(part 1 of 2)
# Autodesk Inventor assembly: HCMUTE-CDT23-PLXR_ASEMBLY
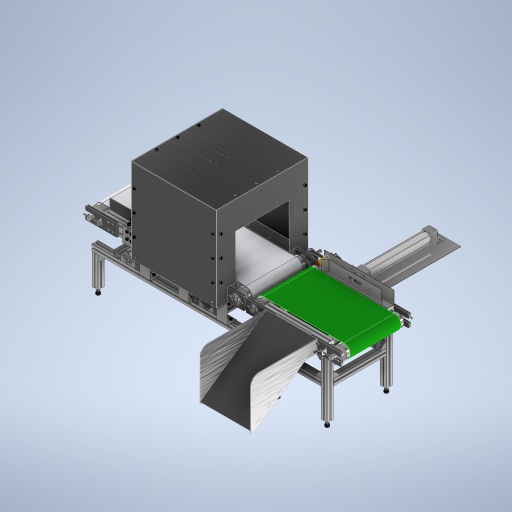
[picture p0: Inventor's stored thumbnail of the model, 512x512]
Saved by Autodesk Inventor 2023 (Build 270158000, 158)
## iProperties
Created: 2023-11-19
Part Number: HCMUTE-CDT23-PLXR_ASEMBLY
Document SubType Name: Assembly
Designer: havie
Mass: 52555 g
Surface Area: 83477.5 cm^2
Volume: 13075.1 cm^3
Density: 4.01946 g/cm^3
Author: havie
## Documents named in this file (82)
- D:\DO_AN_CDT\1.1. PART\HCMUTE-CDT23-PLXR_ASEMBLY.iam
- D:\DO_AN_CDT\1.1. PART\HCMUTE-CDT23-FRAME_ASEMBLY.iam
- D:\DO_AN_CDT\1.1. PART\HCMUTE-CDT23-BAT_TRUC_DAN.ipt
- C:\Users\havie\Documents\Inventor\Content Center Files\R2023\en-US\ISO 4762(2)\ISO 4762 - M6 x 16ISO.ipt
- D:\DO_AN_CDT\1.1. PART\HCMUTE-CDT23-GOI_DO_KFL003.ipt
- D:\DO_AN_CDT\1.1. PART\HCMUTE-CDT23-TRUC_DAN.ipt
- D:\DO_AN_CDT\1.1. PART\HCMUTE-CDT23-BAT_CANG_BANG_TAI.ipt
- D:\DO_AN_CDT\1.1. PART\HCMUTE-CDT23-BAT_TRUC_CANG_TAI.ipt
- C:\Users\havie\Documents\Inventor\Content Center Files\R2023\en-US\ISO 4762(2)\ISO 4762 - M6 x 20ISO.ipt
- D:\DO_AN_CDT\1.1. PART\HCMUTE-CDT23-TRUC_CANG.ipt
- D:\DO_AN_CDT\1.1. PART\HCMUTE-CDT23-M6X80_SUOT.ipt
- C:\Users\havie\Documents\Inventor\Content Center Files\R2023\en-US\ISO 7092\ISO 7092 - ST 6 - 140 HV.ipt
- C:\Users\havie\Documents\Inventor\Content Center Files\R2023\en-US\ISO 4032(2)\ISO 4032 - M6 - ISO.ipt
- D:\DO_AN_CDT\1.1. PART\HCMUTE-CDT23-BELT_PHAN_LOAI.ipt
- C:\Users\havie\Documents\Inventor\Content Center Files\R2023\en-US\ISO 4762(2)\ISO 4762 - M6 x 25ISO.ipt
- C:\Users\havie\Documents\Inventor\Content Center Files\R2023\en-US\ISO 4034(2)\ISO 4034 - M6 - ISO.ipt
- D:\DO_AN_CDT\1.1. PART\HCMUTE-CDT23-LOADCELL.ipt
- D:\DO_AN_CDT\1.1. PART\HCMUTE-CDT23-DE_CHEM_LOADCELL.ipt
- D:\DO_AN_CDT\1.1. PART\HCMUTE-CDT23-DE_GA_LOADCELL.ipt
- D:\DO_AN_CDT\1.1. PART\HCMUTE-CDT23-GOI_CHONG_QTAI.ipt
- D:\DO_AN_CDT\1.1. PART\HCMUTE-CDT23-GOI_DO.ipt
- C:\Users\havie\Documents\Inventor\Content Center Files\R2023\en-US\ISO 4017(1)\ISO 4017 - M6 x 45 - ISO.ipt
- C:\Users\havie\Documents\Inventor\Content Center Files\R2023\en-US\ISO 4762(2)\ISO 4762 - M6 x 10ISO.ipt
- D:\DO_AN_CDT\1.1. PART\HCMUTE-CDT23-BAN_CAN_LOADCELL.ipt
- D:\DO_AN_CDT\1.1. PART\BANG_TAI_CAN\HCMUTE-CDT23-BTC_ASEMBLY.iam
- C:\Users\havie\Documents\Inventor\Content Center Files\R2023\en-US\ISO 4762(2)\ISO 4762 - M5 x 10ISO.ipt
- C:\Users\havie\Documents\Inventor\Content Center Files\R2023\en-US\ISO 4034(2)\ISO 4034 - M5 - ISO.ipt
- D:\DO_AN_CDT\1.1. PART\HCMUTE-CDT23-PULLY_S5M-15X15X8.ipt
- D:\DO_AN_CDT\1.1. PART\HCMUTE-CDT23-PULLY_S5M-30X15X12.ipt
- D:\DO_AN_CDT\1.1. PART\2309HCMUTE-CDT23-BELT_S5M-320X64X15.ipt
- D:\DO_AN_CDT\1.1. PART\HCMUTE-CDT23-MOTOR_DC24V-100RPM-XD42GA775.ipt
- D:\DO_AN_CDT\1.1. PART\2309HCMUTE-CDT23-BELT_S5M-355X71X15.ipt
- D:\DO_AN_CDT\1.1. PART\HCMUTE-CDT23-GA_DC.ipt
- D:\DO_AN_CDT\1.1. PART\HCMUTE-CDT23-OP_GA-CONLAN.ipt
- D:\DO_AN_CDT\1.1. PART\HCMUTE-CDT23-OP_GA-STEP-42.ipt
- D:\DO_AN_CDT\1.1. PART\HCMUTE-CDT23-OP_NDH-2020X500.ipt
- D:\DO_AN_CDT\1.1. PART\HCMUTE-CDT23-OP_STEP-42.ipt
- C:\Users\havie\Documents\Inventor\Content Center Files\R2023\en-US\ISO 4762(2)\ISO 4762 - M6 x 12ISO.ipt
- C:\Users\havie\Documents\Inventor\Content Center Files\R2023\en-US\301818\301818.ipt
- D:\DO_AN_CDT\1.1. PART\HCMUTE-CDT23-OP_TAMLOT.ipt
- C:\Users\havie\Documents\Inventor\Content Center Files\R2023\en-US\ISO 4762(2)\ISO 4762 - M5 x 12ISO.ipt
- D:\DO_AN_CDT\1.1. PART\HCMUTE-CDT23-OP_PULLY-GT2-30X6X5.ipt
- C:\Users\havie\Documents\Inventor\Content Center Files\R2023\en-US\ISO 4762(2)\ISO 4762 - M5 x 8ISO.ipt
- D:\DO_AN_CDT\1.1. PART\HCMUTE-CDT23-OP_RONG-ROC.ipt
- D:\DO_AN_CDT\1.1. PART\HCMUTE-CDT23-OP_V-WHEEL.ipt
- D:\DO_AN_CDT\1.1. PART\HCMUTE-CDT23-OP_BASE-PLATE.ipt
- D:\DO_AN_CDT\1.1. PART\HCMUTE-CDT23-OP_DVCAM.ipt
- D:\DO_AN_CDT\1.1. PART\CAMERA\Assembly_HCMUTE-CDT23-CAMERA_C270Logitech c270 Assembly.iam
- D:\DO_AN_CDT\1.1. PART\HCMUTE-CDT23-OP_RONG-ROC2.ipt
- D:\DO_AN_CDT\1.1. PART\HCMUTE-CDT23-KXL_CHAN-GA.ipt
- D:\DO_AN_CDT\1.1. PART\HCMUTE-CDT23-KXL_A01.ipt
- C:\Users\havie\Documents\Inventor\Content Center Files\R2023\en-US\ISO 4032(2)\ISO 4032 - M5 - ISO.ipt
- D:\DO_AN_CDT\1.1. PART\2309HCMUTE-CDT23-KXL_GA-VUONG.ipt
- D:\DO_AN_CDT\1.1. PART\HCMUTE-CDT23-KXL_A02.ipt
- D:\DO_AN_CDT\1.1. PART\HCMUTE-CDT23-KXL_A03.ipt
- D:\DO_AN_CDT\1.1. PART\HCMUTE-CDT23-KXL_A04.ipt
- D:\DO_AN_CDT\1.1. PART\HCMUTE-CDT23-KXL_A05.ipt
- D:\DO_AN_CDT\1.1. PART\Part_Cylinder\Assembly_HCMUTE-CDT23-CYLINDER-AIRTAC_SC32X300.iam
- D:\DO_AN_CDT\1.1. PART\HCMUTE-CDT23-TAY_GAT.ipt
- D:\DO_AN_CDT\1.1. PART\Part_Cylinder\2309HCMUTE-CDT23-BE_DO.ipt
- D:\DO_AN_CDT\1.1. PART\HCMUTE-CDT23-VND.ipt
- D:\DO_AN_CDT\1.1. PART\Part_Cylinder\2309HCMUTE-CDT23-DO_GA.ipt
- D:\DO_AN_CDT\1.1. PART\HCMUTE-CDT23-BAC_TRUOT.ipt
- D:\DO_AN_CDT\1.1. PART\HCMUTE-CDT23-TRUC_TRUOT.ipt
- D:\DO_AN_CDT\1.1. PART\CBIEN\Assembly_HCMUTE-CDT23-CB_E3F-DS30C4.iam
- D:\DO_AN_CDT\1.1. PART\Part_Contain-Sample\Assembly_HCMUTE-CDT23_BE-TRUOT.iam
- D:\DO_AN_CDT\1.1. PART\HCMUTE-CDT23-BTC-VND.ipt
- D:\DO_AN_CDT\1.1. PART\HCMUTE-CDT23-OP_GA-CONLAN3.ipt
- D:\DO_AN_CDT\1.1. PART\HCMUTE-CDT23-OP_GA-STEP-423.ipt
- D:\DO_AN_CDT\1.1. PART\HCMUTE-CDT23-OP_NDH-2020X5003.ipt
- D:\DO_AN_CDT\1.1. PART\HCMUTE-CDT23-OP_STEP-423.ipt
- D:\DO_AN_CDT\1.1. PART\HCMUTE-CDT23-OP_TAMLOT3.ipt
- D:\DO_AN_CDT\1.1. PART\HCMUTE-CDT23-OP_PULLY-GT2-30X6X53.ipt
- D:\DO_AN_CDT\1.1. PART\HCMUTE-CDT23-OP_RONG-ROC3.ipt
- D:\DO_AN_CDT\1.1. PART\HCMUTE-CDT23-OP_V-WHEEL1.ipt
- D:\DO_AN_CDT\1.1. PART\HCMUTE-CDT23-OP_BASE-PLATE3.ipt
- D:\DO_AN_CDT\1.1. PART\2309HCMUTE-CDT23-KXL_GA-VUONG1.ipt
- D:\DO_AN_CDT\1.1. PART\HCMUTE-CDT23-KXL_A06.ipt
- C:\Users\havie\Documents\Inventor\Content Center Files\R2023\en-US\ISO 4762(2)\ISO 4762 - M4 x 16ISO.ipt
- C:\Users\havie\Documents\Inventor\Content Center Files\R2023\en-US\ISO 4032(2)\ISO 4032 - M4 - ISO.ipt
- D:\DO_AN_CDT\1.1. PART\BANG_TAI_CAN\HCMUTE-CDT23-GOI_DO_KFL003.ipt
- C:\Users\havie\Documents\Inventor\Content Center Files\R2023\en-US\302828\302828.ipt
## Components (366 placed, 80 different names)
1. HCMUTE-CDT23-FRAME_ASEMBLY:1 [sub-assembly] — Mate:1, Flush:1, Flush:2, Mate:18, Mate:19, Mate:20, Mate:21, Flush:5, Mate:33, Mate:35, Mate:36, Mate:37, Mate:38, Mate:40, Mate:42, Flush:6, Mate:73, Mate:84, Flush:8, Flush:9, Mate:92, Flush:12, Mate:102, Flush:13, Mate:152, Flush:16, Mate:153, Flush:18, Mate:154, Flush:20, Mate:185, Mate:186, Mate:190, Mate:206, Flush:30, Flush:32, Flush:35, Mate:276, Flush:52, Mate:277, Mate:282, Mate:283, Mate:284, Mate:285, Mate:320, Flush:63, Mate:321, Mate:322, Mate:323, Mate:399, Flush:73, Mate:402, Mate:498, Mate:499, Flush:96, Mate:500, Mate:501, Flush:97, Mate:502, Mate:503, Flush:98, Mate:504, Mate:505, Flush:99
2. HCMUTE-CDT23-BAT_TRUC_DAN:1 — Mate:1, Flush:1, Flush:2, Mate:7, Mate:8, Mate:9, Mate:74, Mate:75, Mate:76, Mate:77, Mate:194, Mate:196
3. HCMUTE-CDT23-BAT_TRUC_DAN:2 — Mate:190, Mate:191, Mate:192, Mate:193
4. HCMUTE-CDT23-GOI_DO_KFL003:1 — Mate:7, Mate:8, Mate:9, Mate:16, Mate:17, Mate:78, Mate:80
5. HCMUTE-CDT23-GOI_DO_KFL003:2 — Mate:173, Mate:191
6. HCMUTE-CDT23-BAT_CANG_BANG_TAI:1 — Mate:18, Mate:19, Mate:20, Mate:22, Mate:31, Mate:32, Mate:34, Mate:67, Mate:68, Mate:70
7. HCMUTE-CDT23-TRUC_DAN:1 — Mate:16, Mate:17, Mate:72, Mate:155, Mate:172, Mate:174, Mate:189
8. HCMUTE-CDT23-BAT_TRUC_CANG_TAI:1 — Mate:21, Flush:5, Mate:22, Mate:27, Mate:28, Mate:29, Mate:30, Mate:415, Mate:416, Mate:419, Mate:422
9. ISO 4762 M6 x 16:14 — Mate:29, Mate:30
10. ISO 4762 M6 x 16:16 — Mate:27, Mate:28
11. ISO 4762 M6 x 20:1 — Mate:31, Mate:32
12. ISO 4762 M6 x 20:2 — Mate:33, Mate:34
13. HCMUTE-CDT23-BAT_CANG_BANG_TAI:2 — Mate:35, Mate:36, Mate:37, Mate:39, Mate:41, Mate:43, Angle:1, Mate:54, Mate:56, Mate:61, Flush:77
14. ISO 4762 M6 x 20:3 — Mate:38, Mate:39
15. ISO 4762 M6 x 20:4 — Mate:40, Mate:41
16. HCMUTE-CDT23-BAT_TRUC_CANG_TAI:2 — Mate:42, Flush:6, Mate:43, Mate:44, Mate:45, Mate:46, Mate:47, Mate:48, Mate:49, Mate:50, Mate:51, Mate:52, Mate:400
17. ISO 4762 M6 x 16:17 — Mate:44, Mate:50
18. ISO 4762 M6 x 16:18 — Mate:45, Mate:51
19. ISO 4762 M6 x 16:19 — Mate:46, Mate:49
20. ISO 4762 M6 x 16:20 — Mate:47, Mate:48
21. HCMUTE-CDT23-TRUC_CANG:1 — Mate:52, Flush:7, Mate:422
22. HCMUTE-CDT23-M6X80_SUOT:1 — Mate:54, Mate:55, Mate:57, Mate:59, Mate:60
23. ISO 7092 ST 6 - 140 HV:1 — Mate:55, Mate:56, Mate:58
24. ISO 4032 M6:1 — Mate:57, Mate:58, Mate:59
25. ISO 4032 M6:2 — Mate:60, Mate:61
26. HCMUTE-CDT23-M6X80_SUOT:2 — Mate:67, Mate:69
27. ISO 7092 ST 6 - 140 HV:2 — Mate:68
28. ISO 4032 M6:3
29. ISO 4032 M6:5 — Mate:69, Mate:70
30. HCMUTE-CDT23-BELT_PHAN_LOAI:1 — Mate:72, Mate:73
31. ISO 4762 M6 x 25:1 — Mate:74, Mate:75, Mate:79
32. ISO 4762 M6 x 25:2 — Mate:76, Mate:77, Mate:81
33. ISO 4034 M6:1 — Mate:80, Mate:81
34. ISO 4034 M6:2 — Mate:78, Mate:79
35. ISO 4762 M6 x 25:3 — Mate:83, Mate:192
36. ISO 4762 M6 x 25:4 — Mate:82, Mate:193
37. ISO 4034 M6:3 — Mate:82
38. ISO 4034 M6:4 — Mate:83
39. HCMUTE-CDT23-LOADCELL:1 — Mate:88, Mate:89, Mate:90, Mate:94, Mate:95, Mate:96, Mate:97, Flush:14, Mate:113, Mate:114, Mate:115
40. HCMUTE-CDT23-DE_CHEM_LOADCELL:1 — Mate:85, Mate:86, Mate:87, Mate:88, Mate:89, Mate:90
41. HCMUTE-CDT23-DE_GA_LOADCELL:1 — Mate:84, Flush:8, Flush:9, Mate:85, Mate:86, Mate:87, Mate:93, Mate:98, Mate:99, Mate:100, Mate:101, Flush:19
42. HCMUTE-CDT23-GOI_CHONG_QTAI:1 — Mate:102, Flush:13, Mate:103, Mate:104, Flush:14
43. HCMUTE-CDT23-GOI_DO:1 — Mate:92, Flush:12, Mate:93, Mate:105, Mate:106, Mate:107, Mate:108, Mate:109, Mate:110, Mate:111, Mate:112, Flush:17
44. ISO 4017 M6 x 45:1 — Mate:94, Mate:97
45. ISO 4017 M6 x 45:2 — Mate:95, Mate:96
46. ISO 4762 M6 x 16:31 — Mate:100, Mate:101
47. ISO 4762 M6 x 16:33 — Mate:98, Mate:99
48. ISO 4762 M6 x 16:34 — Mate:103, Mate:104
49. ISO 4762 M6 x 10:1 — Mate:105, Mate:106
50. ISO 4762 M6 x 10:2 — Mate:111, Mate:112
51. ISO 4762 M6 x 10:3 — Mate:109, Mate:110
52. ISO 4762 M6 x 10:4 — Mate:107, Mate:108
53. HCMUTE-CDT23-BAN_CAN_LOADCELL:1 — Mate:113, Mate:114, Mate:115, Mate:116, Mate:117, Mate:118, Mate:119, Mate:156, Mate:157, Mate:158, Mate:159, Mate:160, Mate:161, Mate:162, Mate:163
54. ISO 4762 M6 x 25:5 — Mate:116, Mate:118
55. ISO 4762 M6 x 25:6 — Mate:117, Mate:119
56. HCMUTE-CDT23-LOADCELL:2 — Flush:21
57. HCMUTE-CDT23-DE_CHEM_LOADCELL:2
58. HCMUTE-CDT23-DE_GA_LOADCELL:2 — Mate:153, Flush:18, Flush:19
59. HCMUTE-CDT23-GOI_CHONG_QTAI:2 — Mate:154, Flush:20, Flush:21
60. HCMUTE-CDT23-GOI_DO:2 — Mate:152, Flush:16, Flush:17
61. ISO 4017 M6 x 45:3
62. ISO 4017 M6 x 45:4
63. ISO 4762 M6 x 16:35
64. ISO 4762 M6 x 16:36
65. ISO 4762 M6 x 16:37
66. ISO 4762 M6 x 10:5
67. ISO 4762 M6 x 10:6
68. ISO 4762 M6 x 10:7
69. ISO 4762 M6 x 10:8
70. HCMUTE-CDT23-BAN_CAN_LOADCELL:2
71. ISO 4762 M6 x 25:7
72. ISO 4762 M6 x 25:8
73. HCMUTE-CDT23-BTC_ASEMBLY:1 [sub-assembly] — Mate:155, Mate:164, Mate:166, Mate:168, Mate:170, Mate:176, Mate:178, Mate:203, Mate:423, Flush:78, Mate:425, Mate:426, Flush:92, Mate:462, Flush:93, Flush:95, Mate:497
74. HCMUTE-CDT23-PULLY_S5M-30X15X12:1 — Mate:172, Mate:173, Mate:175, Flush:24, Mate:177, Mate:179
75. HCMUTE-CDT23-PULLY_S5M-30X15X12:2 — Mate:174, Mate:175, Flush:25
76. HCMUTE-CDT23-PULLY_S5M-30X15X12:3 — Mate:176, Flush:24
77. 2309HCMUTE-CDT23-BELT_S5M-320X64X15:1 — Mate:177, Mate:178, Mate:179
78. HCMUTE-CDT23-MOTOR_DC24V-100RPM-XD42GA775:1 — Mate:180, Mate:181, Mate:182, Mate:183
79. HCMUTE-CDT23-PULLY_S5M-15X15X8:1 — Mate:183, Mate:184, Flush:25, Mate:187, Mate:188
80. 2309HCMUTE-CDT23-BELT_S5M-355X71X15:1 — Mate:187, Mate:188, Mate:189
81. HCMUTE-CDT23-GA_DC:1 — Mate:180, Mate:181, Mate:182, Mate:184, Mate:185, Mate:186
82. HCMUTE-CDT23-OP_GA-CONLAN:1 — Mate:202, Flush:28, Flush:34, Mate:221, Mate:222, Mate:223, Mate:224, Mate:225, Mate:226, Mate:236
83. HCMUTE-CDT23-OP_GA-STEP-42:1 — Mate:199, Flush:26, Flush:27, Mate:200, Mate:201, Mate:216, Mate:217, Mate:218, Mate:219, Mate:220
84. HCMUTE-CDT23-OP_NDH-2020X500:1 — Mate:199, Flush:26, Flush:27, Mate:202, Flush:28, Mate:203, Flush:31, Mate:208, Mate:210, Flush:34, Flush:35, Flush:39, Flush:40, Mate:426, Flush:80
85. HCMUTE-CDT23-OP_STEP-42:1 — Mate:200, Mate:201, Mate:215
86. ISO 4762 M6 x 12:7
87. ISO 4762 M6 x 12:8
88. ISO 4762 M6 x 12:9
89. ISO 4762 M6 x 12:10
90. ISO 4762 M6 x 12:11
91. ISO 4762 M6 x 12:12
92. 301818 302828.1:1 — Mate:207, Mate:208, Flush:32, Flush:33, Mate:214
93. HCMUTE-CDT23-OP_TAMLOT:1 — Mate:206, Flush:30, Flush:31, Mate:207, Mate:209, Mate:211, Mate:213
94. 301818 302828.1:2 — Mate:209, Mate:210, Flush:33, Mate:212
95. ISO 4762 M5 x 12:1 — Mate:211, Mate:212
96. ISO 4762 M5 x 12:2 — Mate:213, Mate:214
97. HCMUTE-CDT23-OP_PULLY-GT2-30X6X5:1 — Mate:215, Mate:216
98. ISO 4762 M5 x 8:1 — Mate:217, Mate:218
99. ISO 4762 M5 x 8:2 — Mate:219, Mate:220
100. ISO 4762 M5 x 8:3 — Mate:221, Mate:222
101. ISO 4762 M5 x 8:4 — Mate:223, Mate:224
102. HCMUTE-CDT23-OP_RONG-ROC:1 — Mate:225, Mate:226
103. HCMUTE-CDT23-OP_V-WHEEL:1 — Mate:227, Mate:228, Flush:37, Flush:38
104. HCMUTE-CDT23-OP_BASE-PLATE:1 — Mate:227, Mate:228, Mate:229, Mate:230, Mate:231, Mate:232, Mate:233, Mate:234, Angle:3, Mate:236, Flush:80, Mate:427, Mate:428, Angle:9
105. HCMUTE-CDT23-OP_V-WHEEL:3 — Mate:229, Mate:230
106. HCMUTE-CDT23-OP_V-WHEEL:4 — Mate:231, Mate:232
107. HCMUTE-CDT23-OP_V-WHEEL:5 — Mate:233, Mate:234
108. HCMUTE-CDT23-OP_DVCAM:1 — Mate:273, Mate:274, Mate:275, Mate:427, Mate:428, Angle:9
109. Assembly_HCMUTE-CDT23-CAMERA_C270Logitech c270 Assembly:1 [sub-assembly] — Mate:273, Mate:274, Mate:275
110. HCMUTE-CDT23-OP_RONG-ROC2:1
111. HCMUTE-CDT23-KXL_CHAN-GA:1 — Mate:276, Flush:52, Mate:277, Mate:278, Mate:279, Mate:280, Mate:281, Flush:53, Mate:286, Mate:287
112. HCMUTE-CDT23-KXL_CHAN-GA:2 — Mate:282, Mate:283, Flush:53, Flush:54, Flush:65
113. HCMUTE-CDT23-KXL_CHAN-GA:3 — Mate:284, Mate:285, Flush:54, Mate:296, Flush:67
114. HCMUTE-CDT23-KXL_A01:1 — Mate:286, Mate:287, Mate:288, Flush:55, Mate:289, Mate:290, Mate:291, Mate:292, Mate:293, Flush:57, Mate:313, Mate:360
115. 2309HCMUTE-CDT23-KXL_GA-VUONG:1 — Mate:288, Flush:55, Mate:289, Flush:56, Mate:476, Mate:477
116. 2309HCMUTE-CDT23-KXL_GA-VUONG:2 — Mate:290, Flush:56, Mate:291
117. 2309HCMUTE-CDT23-KXL_GA-VUONG:3 — Mate:292, Mate:293, Flush:57, Mate:478
118. ISO 4032 M5:1 — Mate:296
119. HCMUTE-CDT23-KXL_A03:1 — Mate:313, Mate:316, Mate:319, Flush:61, Flush:62, Mate:338, Mate:355, Mate:356, Mate:370, Symmetry:3
120. HCMUTE-CDT23-KXL_A02:2 — Mate:319, Flush:61, Flush:62, Mate:333, Mate:334, Mate:335, Flush:69, Mate:336, Mate:337, Mate:341, Mate:342, Mate:347, Mate:348, Mate:351, Mate:352, Mate:474, Mate:475
121. HCMUTE-CDT23-KXL_CHAN-GA:4 — Mate:320, Flush:63, Mate:321, Flush:64, Flush:66
122. HCMUTE-CDT23-KXL_CHAN-GA:5 — Mate:322, Flush:64, Flush:65, Mate:326
123. HCMUTE-CDT23-KXL_CHAN-GA:6 — Mate:323, Flush:66, Flush:67, Mate:324, Flush:68, Mate:325, Mate:327, Mate:328, Mate:329, Mate:330, Mate:332, Mate:340
124. HCMUTE-CDT23-KXL_A01:2 — Mate:324, Flush:68, Mate:325, Mate:326, Mate:331
125. HCMUTE-CDT23-KXL_A04:1 — Mate:360, Mate:361, Mate:362, Mate:363, Mate:364, Mate:373, Mate:380, Mate:381, Symmetry:3
126. HCMUTE-CDT23-KXL_A05:1 — Mate:370, Mate:371, Flush:72, Mate:372, Mate:374, Mate:375, Mate:382, Mate:383, Mate:384, Mate:385, Mate:386, Mate:481, Mate:482, Mate:483, Mate:484, Mate:485, Mate:486, Mate:487, Mate:488
127. ISO 4762 M5 x 12:44
128. ISO 4032 M5:40
129. ISO 4032 M5:41
130. ISO 4762 M5 x 12:45
131. ISO 4762 M5 x 12:46
132. ISO 4032 M5:42
133. ISO 4032 M5:43
134. ISO 4762 M5 x 12:47
135. ISO 4762 M5 x 12:48
136. ISO 4032 M5:44
137. ISO 4032 M5:45
138. ISO 4762 M5 x 12:49
139. Assembly_HCMUTE-CDT23-CAMERA_C270Logitech c270 Assembly:2 [sub-assembly] — Mate:384, Mate:385, Mate:386, Mate:493, Mate:494, Mate:495, Mate:496
140. Assembly_HCMUTE-CDT23-CYLINDER-AIRTAC_SC32X300:1 [sub-assembly] — Tangent:1, Mate:401, Mate:403, Mate:404, Angle:6, Mate:405, Mate:406, Mate:407
141. HCMUTE-CDT23-TAY_GAT:1 — Tangent:1, Mate:401, Flush:76, Mate:412
142. 2309HCMUTE-CDT23-BE_DO:1 — Mate:399, Flush:73, Mate:400, Flush:74
143. HCMUTE-CDT23-VND:1 — Mate:402, Flush:74, Mate:403, Mate:404, Angle:6, Mate:408, Mate:409, Mate:410, Flush:77, Mate:413, Mate:414
144. 2309HCMUTE-CDT23-DO_GA:1 — Mate:405, Mate:406, Mate:407
145. HCMUTE-CDT23-BAC_TRUOT:1 — Mate:408, Mate:409, Mate:410, Mate:411
146. HCMUTE-CDT23-TRUC_TRUOT:1 — Mate:411, Flush:76, Mate:412
147. Assembly_HCMUTE-CDT23-CB_E3F-DS30C4:1 [sub-assembly] — Mate:413, Mate:414
148. Assembly_HCMUTE-CDT23_BE-TRUOT:1 [sub-assembly] — Angle:7, Angle:8, Mate:415, Mate:416, Mate:417, Mate:418, Mate:419, Mate:420, Mate:421
149. ISO 4762 M6 x 16:38 — Mate:417, Mate:418
150. ISO 4762 M6 x 16:39 — Mate:420, Mate:421
151. HCMUTE-CDT23-BTC-VND:1 — Mate:424, Mate:425, Flush:92, Flush:94, Mate:468
152. HCMUTE-CDT23-OP_GA-CONLAN3:1 — Flush:81, Flush:82, Mate:429, Mate:447, Mate:449, Mate:451, Mate:452, Mate:453
153. HCMUTE-CDT23-OP_GA-STEP-423:1 — Flush:83, Flush:84, Mate:430, Mate:431, Mate:432, Mate:441, Mate:443, Mate:445
154. HCMUTE-CDT23-OP_NDH-2020X5003:1 — Flush:81, Flush:82, Mate:429, Flush:83, Flush:84, Mate:430, Mate:433, Flush:85, Mate:435, Flush:87, Flush:90, Flush:91
155. HCMUTE-CDT23-OP_STEP-423:1 — Mate:431, Mate:432, Mate:442
156. 301818 302828.1:3 — Mate:433, Mate:434, Flush:86, Mate:439
157. HCMUTE-CDT23-OP_TAMLOT3:1 — Mate:434, Flush:85, Mate:436
158. 301818 302828.1:4 — Flush:86, Mate:435, Mate:436, Mate:437
159. ISO 4762 M5 x 12:50 — Mate:437
160. ISO 4762 M5 x 12:51 — Mate:439
161. HCMUTE-CDT23-OP_PULLY-GT2-30X6X53:1 — Mate:441, Mate:442
162. ISO 4762 M5 x 8:5 — Mate:443
163. ISO 4762 M5 x 8:6 — Mate:445
164. ISO 4762 M5 x 8:7 — Mate:447
165. ISO 4762 M5 x 8:8 — Mate:449
166. HCMUTE-CDT23-OP_RONG-ROC3:1 — Mate:451, Mate:452
167. HCMUTE-CDT23-OP_V-WHEEL1:1 — Mate:454, Mate:455, Flush:88, Flush:89
168. HCMUTE-CDT23-OP_BASE-PLATE3:1 — Flush:87, Mate:453, Angle:10, Mate:454, Mate:455, Mate:456, Mate:457, Mate:458, Mate:459, Mate:460, Mate:461
169. HCMUTE-CDT23-OP_V-WHEEL1:2 — Mate:456, Mate:457
170. HCMUTE-CDT23-OP_V-WHEEL1:3 — Mate:458, Mate:459
171. HCMUTE-CDT23-OP_V-WHEEL1:4 — Mate:460, Mate:461
172. HCMUTE-CDT23-BTC-VND:2 — Mate:462, Flush:93, Flush:94
173. 2309HCMUTE-CDT23-KXL_GA-VUONG1:1 — Mate:469, Mate:471
174. 2309HCMUTE-CDT23-KXL_GA-VUONG1:2
175. 2309HCMUTE-CDT23-KXL_GA-VUONG1:3
176. 2309HCMUTE-CDT23-KXL_GA-VUONG1:4
177. 2309HCMUTE-CDT23-KXL_GA-VUONG1:5
178. ISO 4762 M5 x 12:62 — Mate:471, Mate:473
179. ISO 4032 M5:51 — Mate:473
180. ISO 4762 M5 x 12:63 — Mate:469
181. ISO 4762 M5 x 12:64
182. ISO 4032 M5:52
183. ISO 4762 M5 x 12:65
184. ISO 4762 M5 x 12:66
185. ISO 4032 M5:53
186. ISO 4762 M5 x 12:67
187. ISO 4762 M5 x 12:68
188. ISO 4032 M5:54
189. ISO 4762 M5 x 12:69
190. ISO 4762 M5 x 12:70
191. ISO 4032 M5:55
192. ISO 4762 M5 x 12:71
193. Assembly_HCMUTE-CDT23-CB_E3F-DS30C4:2 [sub-assembly] — Mate:474, Mate:475
194. HCMUTE-CDT23-KXL_A06:1 — Mate:476, Mate:477, Mate:478
195. ISO 4032 M5:60 — Mate:479
196. ISO 4032 M5:61 — Mate:480
197. ISO 4762 M5 x 12:76 — Mate:480
198. ISO 4762 M5 x 12:77 — Mate:479
199. ISO 4032 M5:62
200. ISO 4032 M5:63
201. ISO 4762 M5 x 12:78
202. ISO 4762 M5 x 12:79
203. ISO 4032 M5:64
204. ISO 4032 M5:65
205. ISO 4762 M5 x 12:80
206. ISO 4762 M5 x 12:81
207. ISO 4762 M4 x 16:1 — Mate:483, Mate:486, Mate:490
208. ISO 4762 M4 x 16:2 — Mate:482, Mate:487, Mate:489
209. ISO 4762 M4 x 16:3 — Mate:481, Mate:488, Mate:491
210. ISO 4762 M4 x 16:4 — Mate:484, Mate:485, Mate:492
211. ISO 4032 M4:1 — Mate:489, Mate:494
212. ISO 4032 M4:2 — Mate:490, Mate:496
213. ISO 4032 M4:3 — Mate:491, Mate:493
214. ISO 4032 M4:4 — Mate:492, Mate:495
215. HCMUTE-CDT23-GOI_DO_KFL003:3 — Mate:497
216. 302828 302828:1 — Mate:498, Mate:499, Flush:96
217. 302828 302828:2 — Mate:500, Mate:501, Flush:97
218. 302828 302828:3 — Mate:502, Mate:503, Flush:98
219. 302828 302828:4 — Mate:504, Mate:505, Flush:99
220. ISO 4034 M5:2 — Mate:166, Mate:167
221. ISO 4762 M5 x 10:1 — Mate:156, Mate:157, Mate:167
222. ISO 4034 M5:3 — Mate:168, Mate:169
223. ISO 4762 M5 x 10:3 — Mate:160, Mate:161, Mate:169
224. ISO 4034 M5:4 — Mate:170, Mate:171
225. ISO 4034 M5:1 — Mate:164, Mate:165
226. ISO 4762 M5 x 10:4 — Mate:162, Mate:163, Mate:165
227. ISO 4762 M5 x 10:2 — Mate:158, Mate:159, Mate:171
228. ISO 4034 M5:5
229. ISO 4762 M5 x 10:5
230. ISO 4034 M5:6
231. ISO 4762 M5 x 10:6
232. ISO 4034 M5:7
233. ISO 4034 M5:8
234. ISO 4762 M5 x 10:7
235. ISO 4762 M5 x 10:8
236. ISO 4762 M6 x 12:1 — Mate:194
237. ISO 4762 M6 x 12:2 — Mate:196
238. ISO 4762 M6 x 12:3
239. ISO 4762 M6 x 12:4
240. ISO 4762 M6 x 12:5
241. ISO 4762 M6 x 12:6
242. ISO 4762 M6 x 10:9 — Mate:280, Mate:281
243. ISO 4762 M6 x 10:10 — Mate:278, Mate:279
244. ISO 4762 M6 x 10:11
245. ISO 4762 M6 x 10:12
246. ISO 4762 M6 x 10:13
247. ISO 4762 M6 x 10:14
248. ISO 4032 M5:10 — Mate:317, Mate:318
249. ISO 4762 M5 x 12:14 — Mate:315, Mate:316, Mate:318
250. ISO 4032 M5:11
251. ISO 4762 M5 x 12:15
252. ISO 4032 M5:12
253. ISO 4762 M5 x 12:16
254. ISO 4762 M6 x 10:16 — Mate:329, Mate:330
255. ISO 4762 M6 x 10:15 — Mate:327, Mate:328
256. ISO 4762 M6 x 10:17
257. ISO 4762 M6 x 10:18
258. ISO 4762 M6 x 10:19
259. ISO 4762 M6 x 10:20
260. 2309HCMUTE-CDT23-KXL_GA-VUONG:10 — Mate:331, Mate:332, Mate:333, Mate:339, Mate:343, Mate:345
261. 2309HCMUTE-CDT23-KXL_GA-VUONG:13
262. 2309HCMUTE-CDT23-KXL_GA-VUONG:14
263. 2309HCMUTE-CDT23-KXL_GA-VUONG:11 — Mate:334, Mate:335, Flush:69, Mate:349
264. 2309HCMUTE-CDT23-KXL_GA-VUONG:12 — Mate:336, Mate:337, Mate:338, Mate:354, Mate:357
265. 2309HCMUTE-CDT23-KXL_GA-VUONG:15
266. 2309HCMUTE-CDT23-KXL_GA-VUONG:16
267. 2309HCMUTE-CDT23-KXL_GA-VUONG:17 — Mate:367
268. 2309HCMUTE-CDT23-KXL_GA-VUONG:18
269. ISO 4032 M5:15 — Mate:343, Mate:344
270. ISO 4032 M5:16 — Mate:345, Mate:346
271. ISO 4762 M5 x 12:20 — Mate:341, Mate:342, Mate:346
272. ISO 4762 M5 x 12:17 — Mate:339, Mate:340, Mate:344
273. ISO 4032 M5:17
274. ISO 4032 M5:18
275. ISO 4762 M5 x 12:21
276. ISO 4762 M5 x 12:22
277. ISO 4032 M5:19
278. ISO 4032 M5:20
279. ISO 4762 M5 x 12:23
280. ISO 4762 M5 x 12:24
281. ISO 4762 M5 x 12:18 — Mate:347, Mate:348, Mate:350
282. ISO 4032 M5:14 — Mate:349, Mate:350
283. ISO 4762 M5 x 12:25
284. ISO 4032 M5:21
285. ISO 4762 M5 x 12:26
286. ISO 4032 M5:22
287. ISO 4032 M5:13 — Mate:353, Mate:354
288. ISO 4762 M5 x 12:19 — Mate:351, Mate:352, Mate:353
289. ISO 4762 M5 x 12:27 — Mate:355, Mate:356, Mate:358
290. ISO 4032 M5:23 — Mate:357, Mate:358
291. ISO 4032 M5:24
292. ISO 4762 M5 x 12:28
293. ISO 4762 M5 x 12:29
294. ISO 4032 M5:25
295. ISO 4032 M5:26
296. ISO 4762 M5 x 12:30
297. ISO 4762 M5 x 12:31
298. ISO 4032 M5:27
299. ISO 4032 M5:29 — Mate:367, Mate:368
300. ISO 4762 M5 x 12:32 — Mate:361, Mate:362, Mate:368
301. ISO 4032 M5:28 — Mate:365, Mate:366
302. ISO 4762 M5 x 12:33 — Mate:363, Mate:364, Mate:366
303. ISO 4032 M5:30
304. ISO 4762 M5 x 12:34
305. ISO 4032 M5:31
306. ISO 4762 M5 x 12:35
307. ISO 4032 M5:32
308. ISO 4762 M5 x 12:36
309. ISO 4032 M5:33
310. ISO 4762 M5 x 12:37
311. 2309HCMUTE-CDT23-KXL_GA-VUONG:19 — Mate:371, Flush:72, Mate:372
312. 2309HCMUTE-CDT23-KXL_GA-VUONG:20
313. 2309HCMUTE-CDT23-KXL_GA-VUONG:21
314. 2309HCMUTE-CDT23-KXL_GA-VUONG:22 — Mate:373, Mate:374, Mate:375, Mate:376, Mate:377, Mate:378, Mate:379
315. 2309HCMUTE-CDT23-KXL_GA-VUONG:23
316. 2309HCMUTE-CDT23-KXL_GA-VUONG:24
317. ISO 4762 M5 x 12:38 — Mate:380, Mate:381
318. ISO 4032 M5:34 — Mate:376, Mate:377
319. ISO 4032 M5:35 — Mate:378, Mate:379
320. ISO 4762 M5 x 12:39 — Mate:382, Mate:383
321. ISO 4762 M5 x 12:40
322. ISO 4032 M5:36
323. ISO 4032 M5:37
324. ISO 4762 M5 x 12:41
325. ISO 4762 M5 x 12:42
326. ISO 4032 M5:38
327. ISO 4032 M5:39
328. ISO 4762 M5 x 12:43
329. 2309HCMUTE-CDT23-KXL_GA-VUONG:25 — Mate:423, Flush:78, Mate:424, Flush:95, Mate:463, Mate:464, Mate:465, Mate:466
330. 2309HCMUTE-CDT23-KXL_GA-VUONG:26
331. 2309HCMUTE-CDT23-KXL_GA-VUONG:27
332. 2309HCMUTE-CDT23-KXL_GA-VUONG:28
333. 2309HCMUTE-CDT23-KXL_GA-VUONG:29
334. ISO 4762 M5 x 12:53 — Mate:463, Mate:464, Mate:467
335. ISO 4032 M5:46 — Mate:467, Mate:468
336. ISO 4762 M5 x 12:52 — Mate:465, Mate:466
337. ISO 4762 M5 x 12:54
338. ISO 4032 M5:47
339. ISO 4762 M5 x 12:55
340. ISO 4762 M5 x 12:56
341. ISO 4032 M5:48
342. ISO 4762 M5 x 12:57
343. ISO 4762 M5 x 12:58
344. ISO 4032 M5:49
345. ISO 4762 M5 x 12:59
346. ISO 4762 M5 x 12:60
347. ISO 4032 M5:50
348. ISO 4762 M5 x 12:61
349. 2309HCMUTE-CDT23-KXL_GA-VUONG:4 — Mate:309, Mate:365
350. ISO 4032 M5:5 — Mate:309, Mate:310
351. ISO 4762 M5 x 12:8 — Mate:310
352. 2309HCMUTE-CDT23-KXL_GA-VUONG:30
353. ISO 4032 M5:56
354. ISO 4762 M5 x 12:72
355. 2309HCMUTE-CDT23-KXL_GA-VUONG:31
356. ISO 4032 M5:57
357. ISO 4762 M5 x 12:73
358. ISO 4032 M5:4 — Mate:311, Mate:312
359. 2309HCMUTE-CDT23-KXL_GA-VUONG:7 — Mate:312, Mate:315, Mate:317
360. ISO 4762 M5 x 12:9 — Mate:311
361. ISO 4032 M5:58
362. 2309HCMUTE-CDT23-KXL_GA-VUONG:32
363. ISO 4762 M5 x 12:74
364. ISO 4032 M5:59
365. 2309HCMUTE-CDT23-KXL_GA-VUONG:33
366. ISO 4762 M5 x 12:75
## Component patterns: (2 elements, first: ISO 4034 M5:2 + ISO 4762 M5 x 10:1 + ISO 4034 M5:3 + ISO 4762 M5 x 10:3 + ISO 4034 M5:4 + ISO 4034 M5:1 + ISO 4762 M5 x 10:4 + ISO 4762 M5 x 10:2), (3 elements, first: ISO 4762 M6 x 12:1 + ISO 4762 M6 x 12:2), (3 elements, first: ISO 4762 M6 x 10:9 + ISO 4762 M6 x 10:10), (3 elements, first: ISO 4032 M5:10 + ISO 4762 M5 x 12:14), (3 elements, first: ISO 4762 M6 x 10:16 + ISO 4762 M6 x 10:15), (3 elements, first: 2309HCMUTE-CDT23-KXL_GA-VUONG:10), (3 elements, first: 2309HCMUTE-CDT23-KXL_GA-VUONG:11 + 2309HCMUTE-CDT23-KXL_GA-VUONG:12), (3 elements, first: ISO 4032 M5:15 + ISO 4032 M5:16 + ISO 4762 M5 x 12:20 + ISO 4762 M5 x 12:17), (3 elements, first: ISO 4762 M5 x 12:18 + ISO 4032 M5:14), (3 elements, first: ISO 4032 M5:13 + ISO 4762 M5 x 12:19 + ISO 4762 M5 x 12:27 + ISO 4032 M5:23), (3 elements, first: ISO 4032 M5:29 + ISO 4762 M5 x 12:32 + ISO 4032 M5:28 + ISO 4762 M5 x 12:33), (3 elements, first: 2309HCMUTE-CDT23-KXL_GA-VUONG:19), (3 elements, first: 2309HCMUTE-CDT23-KXL_GA-VUONG:22), (3 elements, first: ISO 4762 M5 x 12:38 + ISO 4032 M5:34 + ISO 4032 M5:35 + ISO 4762 M5 x 12:39), (5 elements, first: 2309HCMUTE-CDT23-KXL_GA-VUONG:25), (5 elements, first: ISO 4762 M5 x 12:53 + ISO 4032 M5:46 + ISO 4762 M5 x 12:52), (3 elements, first: 2309HCMUTE-CDT23-KXL_GA-VUONG:4 + ISO 4032 M5:5 + ISO 4762 M5 x 12:8), (3 elements, first: ISO 4032 M5:4 + 2309HCMUTE-CDT23-KXL_GA-VUONG:7 + ISO 4762 M5 x 12:9)
## Relationships (492: Mate 408, Flush 73, Angle 7, Symmetry 3, Tangent 1)
- Mate:1: HCMUTE-CDT23-FRAME_ASEMBLY:1 ↔ HCMUTE-CDT23-BAT_TRUC_DAN:1
- Flush:1: HCMUTE-CDT23-FRAME_ASEMBLY:1 ↔ HCMUTE-CDT23-BAT_TRUC_DAN:1
- Flush:2 (-90 mm): HCMUTE-CDT23-FRAME_ASEMBLY:1 ↔ HCMUTE-CDT23-BAT_TRUC_DAN:1
- Mate:7: HCMUTE-CDT23-BAT_TRUC_DAN:1 ↔ HCMUTE-CDT23-GOI_DO_KFL003:1
- Mate:8: HCMUTE-CDT23-BAT_TRUC_DAN:1 ↔ HCMUTE-CDT23-GOI_DO_KFL003:1
- Mate:9: HCMUTE-CDT23-BAT_TRUC_DAN:1 ↔ HCMUTE-CDT23-GOI_DO_KFL003:1
- Mate:16: HCMUTE-CDT23-GOI_DO_KFL003:1 ↔ HCMUTE-CDT23-TRUC_DAN:1
- Mate:17 (13 mm): HCMUTE-CDT23-GOI_DO_KFL003:1 ↔ HCMUTE-CDT23-TRUC_DAN:1
- Mate:18: HCMUTE-CDT23-FRAME_ASEMBLY:1 ↔ HCMUTE-CDT23-BAT_CANG_BANG_TAI:1
- Mate:19: HCMUTE-CDT23-FRAME_ASEMBLY:1 ↔ HCMUTE-CDT23-BAT_CANG_BANG_TAI:1
- Mate:20: HCMUTE-CDT23-FRAME_ASEMBLY:1 ↔ HCMUTE-CDT23-BAT_CANG_BANG_TAI:1
- Mate:21: HCMUTE-CDT23-FRAME_ASEMBLY:1 ↔ HCMUTE-CDT23-BAT_TRUC_CANG_TAI:1
- Flush:5: HCMUTE-CDT23-FRAME_ASEMBLY:1 ↔ HCMUTE-CDT23-BAT_TRUC_CANG_TAI:1
- Mate:22: HCMUTE-CDT23-BAT_CANG_BANG_TAI:1 ↔ HCMUTE-CDT23-BAT_TRUC_CANG_TAI:1
- Mate:27: HCMUTE-CDT23-BAT_TRUC_CANG_TAI:1 ↔ ISO 4762 M6 x 16:16
- Mate:28: HCMUTE-CDT23-BAT_TRUC_CANG_TAI:1 ↔ ISO 4762 M6 x 16:16
- Mate:29: HCMUTE-CDT23-BAT_TRUC_CANG_TAI:1 ↔ ISO 4762 M6 x 16:14
- Mate:30: HCMUTE-CDT23-BAT_TRUC_CANG_TAI:1 ↔ ISO 4762 M6 x 16:14
- Mate:31: HCMUTE-CDT23-BAT_CANG_BANG_TAI:1 ↔ ISO 4762 M6 x 20:1
- Mate:32: HCMUTE-CDT23-BAT_CANG_BANG_TAI:1 ↔ ISO 4762 M6 x 20:1
- Mate:33: HCMUTE-CDT23-FRAME_ASEMBLY:1 ↔ ISO 4762 M6 x 20:2
- Mate:34: HCMUTE-CDT23-BAT_CANG_BANG_TAI:1 ↔ ISO 4762 M6 x 20:2
- Mate:35: HCMUTE-CDT23-FRAME_ASEMBLY:1 ↔ HCMUTE-CDT23-BAT_CANG_BANG_TAI:2
- Mate:36: HCMUTE-CDT23-FRAME_ASEMBLY:1 ↔ HCMUTE-CDT23-BAT_CANG_BANG_TAI:2
- Mate:37: HCMUTE-CDT23-FRAME_ASEMBLY:1 ↔ HCMUTE-CDT23-BAT_CANG_BANG_TAI:2
- Mate:38: HCMUTE-CDT23-FRAME_ASEMBLY:1 ↔ ISO 4762 M6 x 20:3
- Mate:39: HCMUTE-CDT23-BAT_CANG_BANG_TAI:2 ↔ ISO 4762 M6 x 20:3
- Mate:40: HCMUTE-CDT23-FRAME_ASEMBLY:1 ↔ ISO 4762 M6 x 20:4
- Mate:41: HCMUTE-CDT23-BAT_CANG_BANG_TAI:2 ↔ ISO 4762 M6 x 20:4
- Mate:42: HCMUTE-CDT23-FRAME_ASEMBLY:1 ↔ HCMUTE-CDT23-BAT_TRUC_CANG_TAI:2
- Flush:6: HCMUTE-CDT23-FRAME_ASEMBLY:1 ↔ HCMUTE-CDT23-BAT_TRUC_CANG_TAI:2
- Mate:43: HCMUTE-CDT23-BAT_CANG_BANG_TAI:2 ↔ HCMUTE-CDT23-BAT_TRUC_CANG_TAI:2
- Mate:44: HCMUTE-CDT23-BAT_TRUC_CANG_TAI:2 ↔ ISO 4762 M6 x 16:17
- Mate:45: HCMUTE-CDT23-BAT_TRUC_CANG_TAI:2 ↔ ISO 4762 M6 x 16:18
- Mate:46: HCMUTE-CDT23-BAT_TRUC_CANG_TAI:2 ↔ ISO 4762 M6 x 16:19
- Mate:47: HCMUTE-CDT23-BAT_TRUC_CANG_TAI:2 ↔ ISO 4762 M6 x 16:20
- Mate:48: HCMUTE-CDT23-BAT_TRUC_CANG_TAI:2 ↔ ISO 4762 M6 x 16:20
- Mate:49: HCMUTE-CDT23-BAT_TRUC_CANG_TAI:2 ↔ ISO 4762 M6 x 16:19
- Mate:50: HCMUTE-CDT23-BAT_TRUC_CANG_TAI:2 ↔ ISO 4762 M6 x 16:17
- Mate:51: HCMUTE-CDT23-BAT_TRUC_CANG_TAI:2 ↔ ISO 4762 M6 x 16:18
- Mate:52: HCMUTE-CDT23-BAT_TRUC_CANG_TAI:2 ↔ HCMUTE-CDT23-TRUC_CANG:1
- Angle:1 (0 deg): HCMUTE-CDT23-BAT_CANG_BANG_TAI:2
- Flush:7: HCMUTE-CDT23-TRUC_CANG:1
- Mate:54: HCMUTE-CDT23-BAT_CANG_BANG_TAI:2 ↔ HCMUTE-CDT23-M6X80_SUOT:1
- Mate:55: HCMUTE-CDT23-M6X80_SUOT:1 ↔ ISO 7092 ST 6 - 140 HV:1
- Mate:56: HCMUTE-CDT23-BAT_CANG_BANG_TAI:2 ↔ ISO 7092 ST 6 - 140 HV:1
- Mate:57: HCMUTE-CDT23-M6X80_SUOT:1 ↔ ISO 4032 M6:1
- Mate:58: ISO 7092 ST 6 - 140 HV:1 ↔ ISO 4032 M6:1
- Mate:59: HCMUTE-CDT23-M6X80_SUOT:1 ↔ ISO 4032 M6:1
- Mate:60: HCMUTE-CDT23-M6X80_SUOT:1 ↔ ISO 4032 M6:2
- Mate:61 (24 mm): HCMUTE-CDT23-BAT_CANG_BANG_TAI:2 ↔ ISO 4032 M6:2
- [Mate]: HCMUTE-CDT23-M6X80_SUOT:2 ↔ ISO 7092 ST 6 - 140 HV:2
- [Mate]: HCMUTE-CDT23-M6X80_SUOT:2 ↔ ISO 4032 M6:3
- [Mate]: ISO 7092 ST 6 - 140 HV:2 ↔ ISO 4032 M6:3
- [Mate]: HCMUTE-CDT23-M6X80_SUOT:2 ↔ ISO 4032 M6:3
- Mate:67: HCMUTE-CDT23-BAT_CANG_BANG_TAI:1 ↔ HCMUTE-CDT23-M6X80_SUOT:2
- Mate:68: HCMUTE-CDT23-BAT_CANG_BANG_TAI:1 ↔ ISO 7092 ST 6 - 140 HV:2
- Mate:69: HCMUTE-CDT23-M6X80_SUOT:2 ↔ ISO 4032 M6:5
- Mate:70 (24 mm): HCMUTE-CDT23-BAT_CANG_BANG_TAI:1 ↔ ISO 4032 M6:5
- Mate:72: HCMUTE-CDT23-TRUC_DAN:1 ↔ HCMUTE-CDT23-BELT_PHAN_LOAI:1
- Mate:73 (5 mm): HCMUTE-CDT23-FRAME_ASEMBLY:1 ↔ HCMUTE-CDT23-BELT_PHAN_LOAI:1
- Mate:74: HCMUTE-CDT23-BAT_TRUC_DAN:1 ↔ ISO 4762 M6 x 25:1
- Mate:75: HCMUTE-CDT23-BAT_TRUC_DAN:1 ↔ ISO 4762 M6 x 25:1
- Mate:76: HCMUTE-CDT23-BAT_TRUC_DAN:1 ↔ ISO 4762 M6 x 25:2
- Mate:77: HCMUTE-CDT23-BAT_TRUC_DAN:1 ↔ ISO 4762 M6 x 25:2
- Mate:78: HCMUTE-CDT23-GOI_DO_KFL003:1 ↔ ISO 4034 M6:2
- Mate:79: ISO 4762 M6 x 25:1 ↔ ISO 4034 M6:2
- Mate:80: HCMUTE-CDT23-GOI_DO_KFL003:1 ↔ ISO 4034 M6:1
- Mate:81: ISO 4762 M6 x 25:2 ↔ ISO 4034 M6:1
- Mate:82: ISO 4762 M6 x 25:4 ↔ ISO 4034 M6:3
- Mate:83: ISO 4762 M6 x 25:3 ↔ ISO 4034 M6:4
- Mate:84: HCMUTE-CDT23-FRAME_ASEMBLY:1 ↔ HCMUTE-CDT23-DE_GA_LOADCELL:1
- Flush:8: HCMUTE-CDT23-FRAME_ASEMBLY:1 ↔ HCMUTE-CDT23-DE_GA_LOADCELL:1
- Flush:9 (115 mm): HCMUTE-CDT23-FRAME_ASEMBLY:1 ↔ HCMUTE-CDT23-DE_GA_LOADCELL:1
- Mate:85: HCMUTE-CDT23-DE_CHEM_LOADCELL:1 ↔ HCMUTE-CDT23-DE_GA_LOADCELL:1
- Mate:86: HCMUTE-CDT23-DE_CHEM_LOADCELL:1 ↔ HCMUTE-CDT23-DE_GA_LOADCELL:1
- Mate:87: HCMUTE-CDT23-DE_CHEM_LOADCELL:1 ↔ HCMUTE-CDT23-DE_GA_LOADCELL:1
- Mate:88: HCMUTE-CDT23-LOADCELL:1 ↔ HCMUTE-CDT23-DE_CHEM_LOADCELL:1
- Mate:89: HCMUTE-CDT23-LOADCELL:1 ↔ HCMUTE-CDT23-DE_CHEM_LOADCELL:1
- Mate:90: HCMUTE-CDT23-LOADCELL:1 ↔ HCMUTE-CDT23-DE_CHEM_LOADCELL:1
- Mate:92: HCMUTE-CDT23-FRAME_ASEMBLY:1 ↔ HCMUTE-CDT23-GOI_DO:1
- Flush:12: HCMUTE-CDT23-FRAME_ASEMBLY:1 ↔ HCMUTE-CDT23-GOI_DO:1
- Mate:93: HCMUTE-CDT23-DE_GA_LOADCELL:1 ↔ HCMUTE-CDT23-GOI_DO:1
- Mate:94: HCMUTE-CDT23-LOADCELL:1 ↔ ISO 4017 M6 x 45:1
- Mate:95: HCMUTE-CDT23-LOADCELL:1 ↔ ISO 4017 M6 x 45:2
- Mate:96: HCMUTE-CDT23-LOADCELL:1 ↔ ISO 4017 M6 x 45:2
- Mate:97: HCMUTE-CDT23-LOADCELL:1 ↔ ISO 4017 M6 x 45:1
- Mate:98: HCMUTE-CDT23-DE_GA_LOADCELL:1 ↔ ISO 4762 M6 x 16:33
- Mate:99: HCMUTE-CDT23-DE_GA_LOADCELL:1 ↔ ISO 4762 M6 x 16:33
- Mate:100: HCMUTE-CDT23-DE_GA_LOADCELL:1 ↔ ISO 4762 M6 x 16:31
- Mate:101: HCMUTE-CDT23-DE_GA_LOADCELL:1 ↔ ISO 4762 M6 x 16:31
- Mate:102: HCMUTE-CDT23-FRAME_ASEMBLY:1 ↔ HCMUTE-CDT23-GOI_CHONG_QTAI:1
- Flush:13: HCMUTE-CDT23-FRAME_ASEMBLY:1 ↔ HCMUTE-CDT23-GOI_CHONG_QTAI:1
- Mate:103: HCMUTE-CDT23-GOI_CHONG_QTAI:1 ↔ ISO 4762 M6 x 16:34
- Mate:104: HCMUTE-CDT23-GOI_CHONG_QTAI:1 ↔ ISO 4762 M6 x 16:34
- Flush:14 (-1.5 mm): HCMUTE-CDT23-LOADCELL:1 ↔ HCMUTE-CDT23-GOI_CHONG_QTAI:1
- Mate:105: HCMUTE-CDT23-GOI_DO:1 ↔ ISO 4762 M6 x 10:1
- Mate:106: HCMUTE-CDT23-GOI_DO:1 ↔ ISO 4762 M6 x 10:1
- Mate:107: HCMUTE-CDT23-GOI_DO:1 ↔ ISO 4762 M6 x 10:4
- Mate:108: HCMUTE-CDT23-GOI_DO:1 ↔ ISO 4762 M6 x 10:4
- Mate:109: HCMUTE-CDT23-GOI_DO:1 ↔ ISO 4762 M6 x 10:3
- Mate:110: HCMUTE-CDT23-GOI_DO:1 ↔ ISO 4762 M6 x 10:3
- Mate:111: HCMUTE-CDT23-GOI_DO:1 ↔ ISO 4762 M6 x 10:2
- Mate:112: HCMUTE-CDT23-GOI_DO:1 ↔ ISO 4762 M6 x 10:2
- Mate:113: HCMUTE-CDT23-LOADCELL:1 ↔ HCMUTE-CDT23-BAN_CAN_LOADCELL:1
- Mate:114: HCMUTE-CDT23-LOADCELL:1 ↔ HCMUTE-CDT23-BAN_CAN_LOADCELL:1
- Mate:115: HCMUTE-CDT23-LOADCELL:1 ↔ HCMUTE-CDT23-BAN_CAN_LOADCELL:1
- Mate:116: HCMUTE-CDT23-BAN_CAN_LOADCELL:1 ↔ ISO 4762 M6 x 25:5
- Mate:117: HCMUTE-CDT23-BAN_CAN_LOADCELL:1 ↔ ISO 4762 M6 x 25:6
- Mate:118: HCMUTE-CDT23-BAN_CAN_LOADCELL:1 ↔ ISO 4762 M6 x 25:5
- Mate:119: HCMUTE-CDT23-BAN_CAN_LOADCELL:1 ↔ ISO 4762 M6 x 25:6
- [Mate]: HCMUTE-CDT23-DE_CHEM_LOADCELL:2 ↔ HCMUTE-CDT23-DE_GA_LOADCELL:2
- [Mate]: HCMUTE-CDT23-DE_CHEM_LOADCELL:2 ↔ HCMUTE-CDT23-DE_GA_LOADCELL:2
- [Mate]: HCMUTE-CDT23-DE_CHEM_LOADCELL:2 ↔ HCMUTE-CDT23-DE_GA_LOADCELL:2
- [Mate]: HCMUTE-CDT23-LOADCELL:2 ↔ HCMUTE-CDT23-DE_CHEM_LOADCELL:2
- [Mate]: HCMUTE-CDT23-LOADCELL:2 ↔ HCMUTE-CDT23-DE_CHEM_LOADCELL:2
- [Mate]: HCMUTE-CDT23-LOADCELL:2 ↔ HCMUTE-CDT23-DE_CHEM_LOADCELL:2
- [Mate]: HCMUTE-CDT23-DE_GA_LOADCELL:2 ↔ HCMUTE-CDT23-GOI_DO:2
- [Mate]: HCMUTE-CDT23-LOADCELL:2 ↔ ISO 4017 M6 x 45:3
- [Mate]: HCMUTE-CDT23-LOADCELL:2 ↔ ISO 4017 M6 x 45:4
- [Mate]: HCMUTE-CDT23-LOADCELL:2 ↔ ISO 4017 M6 x 45:4
- [Mate]: HCMUTE-CDT23-LOADCELL:2 ↔ ISO 4017 M6 x 45:3
- [Mate]: HCMUTE-CDT23-DE_GA_LOADCELL:2 ↔ ISO 4762 M6 x 16:36
- [Mate]: HCMUTE-CDT23-DE_GA_LOADCELL:2 ↔ ISO 4762 M6 x 16:36
- [Mate]: HCMUTE-CDT23-DE_GA_LOADCELL:2 ↔ ISO 4762 M6 x 16:35
- [Mate]: HCMUTE-CDT23-DE_GA_LOADCELL:2 ↔ ISO 4762 M6 x 16:35
- [Mate]: HCMUTE-CDT23-GOI_CHONG_QTAI:2 ↔ ISO 4762 M6 x 16:37
- [Mate]: HCMUTE-CDT23-GOI_CHONG_QTAI:2 ↔ ISO 4762 M6 x 16:37
- [Flush] (-1.5 mm): HCMUTE-CDT23-LOADCELL:2 ↔ HCMUTE-CDT23-GOI_CHONG_QTAI:2
- [Mate]: HCMUTE-CDT23-GOI_DO:2 ↔ ISO 4762 M6 x 10:5
- [Mate]: HCMUTE-CDT23-GOI_DO:2 ↔ ISO 4762 M6 x 10:5
- [Mate]: HCMUTE-CDT23-GOI_DO:2 ↔ ISO 4762 M6 x 10:8
- [Mate]: HCMUTE-CDT23-GOI_DO:2 ↔ ISO 4762 M6 x 10:8
- [Mate]: HCMUTE-CDT23-GOI_DO:2 ↔ ISO 4762 M6 x 10:7
- [Mate]: HCMUTE-CDT23-GOI_DO:2 ↔ ISO 4762 M6 x 10:7
- [Mate]: HCMUTE-CDT23-GOI_DO:2 ↔ ISO 4762 M6 x 10:6
- [Mate]: HCMUTE-CDT23-GOI_DO:2 ↔ ISO 4762 M6 x 10:6
- [Mate]: HCMUTE-CDT23-LOADCELL:2 ↔ HCMUTE-CDT23-BAN_CAN_LOADCELL:2
- [Mate]: HCMUTE-CDT23-LOADCELL:2 ↔ HCMUTE-CDT23-BAN_CAN_LOADCELL:2
- [Mate]: HCMUTE-CDT23-LOADCELL:2 ↔ HCMUTE-CDT23-BAN_CAN_LOADCELL:2
- [Mate]: HCMUTE-CDT23-BAN_CAN_LOADCELL:2 ↔ ISO 4762 M6 x 25:7
- [Mate]: HCMUTE-CDT23-BAN_CAN_LOADCELL:2 ↔ ISO 4762 M6 x 25:8
- [Mate]: HCMUTE-CDT23-BAN_CAN_LOADCELL:2 ↔ ISO 4762 M6 x 25:7
- [Mate]: HCMUTE-CDT23-BAN_CAN_LOADCELL:2 ↔ ISO 4762 M6 x 25:8
- Mate:152: HCMUTE-CDT23-FRAME_ASEMBLY:1 ↔ HCMUTE-CDT23-GOI_DO:2
- Flush:16: HCMUTE-CDT23-FRAME_ASEMBLY:1 ↔ HCMUTE-CDT23-GOI_DO:2
- Flush:17: HCMUTE-CDT23-GOI_DO:1 ↔ HCMUTE-CDT23-GOI_DO:2
- Mate:153: HCMUTE-CDT23-FRAME_ASEMBLY:1 ↔ HCMUTE-CDT23-DE_GA_LOADCELL:2
- Flush:18: HCMUTE-CDT23-FRAME_ASEMBLY:1 ↔ HCMUTE-CDT23-DE_GA_LOADCELL:2
- Flush:19: HCMUTE-CDT23-DE_GA_LOADCELL:1 ↔ HCMUTE-CDT23-DE_GA_LOADCELL:2
- Mate:154: HCMUTE-CDT23-FRAME_ASEMBLY:1 ↔ HCMUTE-CDT23-GOI_CHONG_QTAI:2
- Flush:20: HCMUTE-CDT23-FRAME_ASEMBLY:1 ↔ HCMUTE-CDT23-GOI_CHONG_QTAI:2
- Flush:21 (-1.5 mm): HCMUTE-CDT23-LOADCELL:2 ↔ HCMUTE-CDT23-GOI_CHONG_QTAI:2
- Mate:155 (85 mm): HCMUTE-CDT23-TRUC_DAN:1 ↔ HCMUTE-CDT23-BTC_ASEMBLY:1
- Mate:156: HCMUTE-CDT23-BAN_CAN_LOADCELL:1 ↔ ISO 4762 M5 x 10:1
- Mate:157: HCMUTE-CDT23-BAN_CAN_LOADCELL:1 ↔ ISO 4762 M5 x 10:1
- Mate:158: HCMUTE-CDT23-BAN_CAN_LOADCELL:1 ↔ ISO 4762 M5 x 10:2
- Mate:159: HCMUTE-CDT23-BAN_CAN_LOADCELL:1 ↔ ISO 4762 M5 x 10:2
- Mate:160: HCMUTE-CDT23-BAN_CAN_LOADCELL:1 ↔ ISO 4762 M5 x 10:3
- Mate:161: HCMUTE-CDT23-BAN_CAN_LOADCELL:1 ↔ ISO 4762 M5 x 10:3
- Mate:162: HCMUTE-CDT23-BAN_CAN_LOADCELL:1 ↔ ISO 4762 M5 x 10:4
- Mate:163: HCMUTE-CDT23-BAN_CAN_LOADCELL:1 ↔ ISO 4762 M5 x 10:4
- Mate:164: HCMUTE-CDT23-BTC_ASEMBLY:1 ↔ ISO 4034 M5:1
- Mate:165: ISO 4034 M5:1 ↔ ISO 4762 M5 x 10:4
- Mate:166: HCMUTE-CDT23-BTC_ASEMBLY:1 ↔ ISO 4034 M5:2
- Mate:167: ISO 4034 M5:2 ↔ ISO 4762 M5 x 10:1
- Mate:168: HCMUTE-CDT23-BTC_ASEMBLY:1 ↔ ISO 4034 M5:3
- Mate:169: ISO 4034 M5:3 ↔ ISO 4762 M5 x 10:3
- Mate:170: HCMUTE-CDT23-BTC_ASEMBLY:1 ↔ ISO 4034 M5:4
- Mate:171: ISO 4034 M5:4 ↔ ISO 4762 M5 x 10:2
- Mate:172: HCMUTE-CDT23-TRUC_DAN:1 ↔ HCMUTE-CDT23-PULLY_S5M-30X15X12:1
- Mate:173 (10 mm): HCMUTE-CDT23-GOI_DO_KFL003:2 ↔ HCMUTE-CDT23-PULLY_S5M-30X15X12:1
- Mate:174: HCMUTE-CDT23-TRUC_DAN:1 ↔ HCMUTE-CDT23-PULLY_S5M-30X15X12:2
- Mate:175 (10 mm): HCMUTE-CDT23-PULLY_S5M-30X15X12:1 ↔ HCMUTE-CDT23-PULLY_S5M-30X15X12:2
- Mate:176: HCMUTE-CDT23-BTC_ASEMBLY:1 ↔ HCMUTE-CDT23-PULLY_S5M-30X15X12:3
- Flush:24: HCMUTE-CDT23-PULLY_S5M-30X15X12:1 ↔ HCMUTE-CDT23-PULLY_S5M-30X15X12:3